# Autodesk Inventor assembly: SlotAssembly
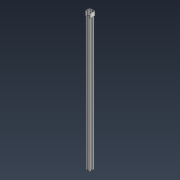
[picture p0: Inventor's stored thumbnail of the model, 180x180]
Saved by Autodesk Inventor 2022 (Build 260153000, 153)
## iProperties
Created: 2022-06-24
Part Number: SlotAssembly
Document SubType Name: Assembly
Designer: tecware
Author: tecware
## Documents named in this file (3)
- C:\Users\tecware\Documents\git\calibrationKit\calibrationKit_v2\l-frame\slotAssembly.iam
- C:\Users\tecware\Documents\git\calibrationKit\calibrationKit_v2\l-frame\slot_test.ipt
- C:\Users\tecware\Documents\git\calibrationKit\calibrationKit_v2\l-frame\components_l-frame\2020 Aluminum profile - 590mm.ipt
## Components (2 placed, 2 different names)
1. slot_test:1 — Insert:1, Mate:1
2. 2020 Aluminum profile - 590mm:1 — Insert:1, Mate:1
## Relationships (2: Insert 1, Mate 1)
- Insert:1: slot_test:1 ↔ 2020 Aluminum profile - 590mm:1
- Mate:1: slot_test:1 ↔ 2020 Aluminum profile - 590mm:1
